# Autodesk Inventor assembly: Assembly1
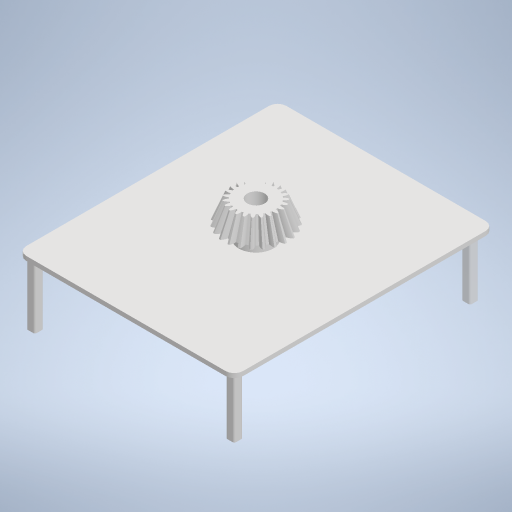
[picture p0: Inventor's stored thumbnail of the model, 512x512]
Saved by Autodesk Inventor 2024 (Build 280153000, 153)
## iProperties
Created: 2023-05-18
Part Number: Assembly1
Document SubType Name: Assembly
Designer: shraa
Author: shraa
## Documents named in this file (4)
- C:\Users\shraa\OneDrive\Documents\explo\Assembly1.iam
- C:\Users\shraa\OneDrive\Documents\explo\Part1.ipt
- C:\Users\shraa\OneDrive\Documents\explo\Part2.ipt
- C:\Users\shraa\OneDrive\Documents\explo\bevel.ipt
## Components (6 placed, 3 different names)
1. Part1:1 — Rotational:1, Rotational:2, Rigid:1, Rigid:2, Rigid:3
2. Part2:1 — Rotational:1
3. Part2:2 — Rotational:2
4. Part2:3 — Rigid:2
5. Part2:4 — Rigid:1
6. bevel:1 — Rigid:3
## Relationships (5: WeldJoint 3, RevoluteJoint 2)
- Rotational:1 [RevoluteJoint]: Part1:1 ↔ Part2:1
- Rotational:2 [RevoluteJoint]: Part1:1 ↔ Part2:2
- Rigid:1 [WeldJoint]: Part1:1 ↔ Part2:4
- Rigid:2 [WeldJoint]: Part1:1 ↔ Part2:3
- Rigid:3 [WeldJoint]: Part1:1 ↔ bevel:1
